# Autodesk Inventor assembly: P1704_EG
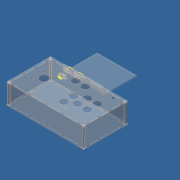
[picture p0: Inventor's stored thumbnail of the model, 180x180]
Saved by Autodesk Inventor 2015 SP2 (Build 190223200, 223)
## iProperties
Created: 2018-05-15
Part Number: P1704_EG
Project: Manette arcade
Description: Manette arcade
Document SubType Name: Assembly
Designer: Alexandre.PICOTTE
Author: Alexandre.PICOTTE
## Documents named in this file (3)
- C:\Users\Alexandre.PICOTTE\Documents\P1704_Manettes\06_Dessins\Manette_arcade\P1704_EG_Manette_arcade.iam
- C:\Users\Alexandre.PICOTTE\Documents\P1704_Manettes\06_Dessins\Manette_arcade\P1704_E1_Manette.iam
- C:\Users\Alexandre.PICOTTE\Documents\P1704_Manettes\06_Dessins\Manette_arcade\P1704_E2_Console.iam
## Components (2 placed, 2 different names)
1. P1704_E1_Manette:1 [sub-assembly] — Affleurement:1, Affleurement:2, Placage:1
2. P1704_E2_Console:1 [sub-assembly] — Affleurement:1, Affleurement:2, Placage:1
## Relationships (3: Flush 2, Mate 1)
- Affleurement:1 [Flush]: P1704_E1_Manette:1 ↔ P1704_E2_Console:1
- Affleurement:2 [Flush]: P1704_E1_Manette:1 ↔ P1704_E2_Console:1
- Placage:1 [Mate] (50 mm): P1704_E1_Manette:1 ↔ P1704_E2_Console:1
